# Autodesk Inventor assembly: Ensamble inicial_ IMPRESION_3D
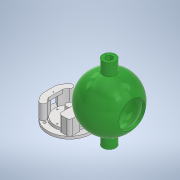
[picture p0: Inventor's stored thumbnail of the model, 180x180]
Saved by Autodesk Inventor 2020.1 (Build 241239000, 239)
## iProperties
Created: 2019-12-10
Part Number: Ensamble inicial_ IMPRESION_3D
Document SubType Name: Assembly
Designer: Daniel
Author: Daniel
## Documents named in this file (4)
- F:\Proyectos\Dog Feeder\Solido\Ensamble Inicial\Ensamble inicial_ IMPRESION_3D.iam
- F:\Proyectos\Dog Feeder\Solido\Ensamble Inicial\Dosificador.ipt
- F:\Proyectos\Dog Feeder\Solido\Ensamble Inicial\Exagono.ipt
- F:\Proyectos\Dog Feeder\Solido\Ensamble Inicial\Soporte_Servo.ipt
## Components (3 placed, 3 different names)
1. Dosificador:1 — Mate:1, Tangent:1, Mate:5
2. Exagono:1 — Mate:2, Mate:4
3. Soporte_Servo:1 — Mate:3, Mate:4, Tangent:1, Mate:6
## Relationships (7: Mate 6, Tangent 1)
- Mate:1: Dosificador:1
- Mate:2: Exagono:1
- Mate:3: Soporte_Servo:1
- Mate:4: Exagono:1 ↔ Soporte_Servo:1
- Tangent:1 (20 mm): Dosificador:1 ↔ Soporte_Servo:1
- Mate:5: Dosificador:1
- Mate:6: Soporte_Servo:1
